# Autodesk Inventor assembly: Chasis_03
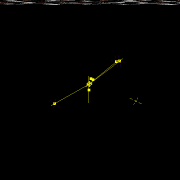
[picture p0: Inventor's stored thumbnail of the model, 180x180]
Saved by Autodesk Inventor 2017 (Build 210142000, 142)
## iProperties
Created: 2017-01-10
Part Number: Chasis_03
Document SubType Name: Assembly
Designer: David Kopala
Author: David Kopala
## Documents named in this file (3)
- \\Mac\Home\Documents\Drone\Drone\3D Models\Project\Chasis_03\Chasis_03.iam
- \\Mac\Home\Documents\Drone\Drone\3D Models\Project\Chasis_03\Outer_Shell.ipt
- \\Mac\Home\Documents\Drone\Drone\3D Models\Project\Chasis_03\BevelSystem.iam
## Components (2 placed, 2 different names)
1. Outer_Shell:1 — Insert:1
2. BevelSystem:1 [sub-assembly] — Insert:1
## Relationships (1: Insert 1)
- Insert:1: Outer_Shell:1 ↔ BevelSystem:1
